# Autodesk Inventor assembly: boltnuttopassembly_MIR
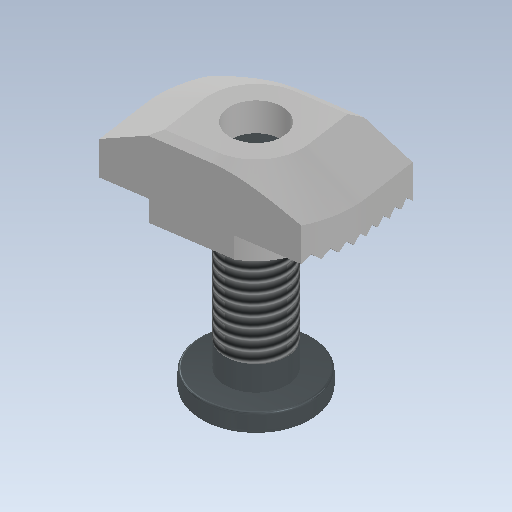
[picture p0: Inventor's stored thumbnail of the model, 512x512]
Saved by Autodesk Inventor 2020.2 (Build 242310000, 310)
## iProperties
Created: 2020-07-25
Part Number: boltnuttopassembly_MIR
Document SubType Name: Assembly
Designer: JK
Author: JK
## Documents named in this file (3)
- C:\Users\JK\Documents\Inventor\Mesa\boltnuttopassembly_MIR.iam
- C:\Users\JK\Documents\Inventor\Mesa\M5x15BoltFlatHead_MIR.ipt
- C:\Users\JK\Documents\Inventor\Mesa\T_Slot_Nut_Dropin_3030m5ipt_MIR.ipt
## Components (2 placed, 2 different names)
1. M5x15BoltFlatHead_MIR:1 — Mate:2, Angle:1, Mate:1
2. T_Slot_Nut_Dropin_3030m5ipt_MIR:1 — Mate:2, Angle:1, Mate:1
## Relationships (3: Mate 2, Angle 1)
- Mate:2 (12.5 mm): M5x15BoltFlatHead_MIR:1 ↔ T_Slot_Nut_Dropin_3030m5ipt_MIR:1
- Angle:1 (0 deg): M5x15BoltFlatHead_MIR:1 ↔ T_Slot_Nut_Dropin_3030m5ipt_MIR:1
- Mate:1: M5x15BoltFlatHead_MIR:1 ↔ T_Slot_Nut_Dropin_3030m5ipt_MIR:1
